(part 1 of 2)
# Autodesk Inventor assembly: 110033226_iam_04_大橋塔樓
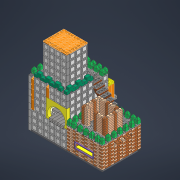
[picture p0: Inventor's stored thumbnail of the model, 180x180]
Saved by Autodesk Inventor 2022 (Build 260153000, 153)
## iProperties
Created: 2022-06-23
Part Number: 110033226_iam_04_大橋塔樓
Document SubType Name: Assembly
Designer: User
Author: User
## Documents named in this file (16)
- D:\D-disk\pomelo\大一\下學期\機械設計製圖\1100332260_LEGOproj_沒有公主城堡\110033226_iam_04_大橋塔樓.iam
- D:\D-disk\pomelo\大一\下學期\機械設計製圖\1100332260_LEGOproj_沒有公主城堡\110033226_ipt_07_磚塊樺木(2x1).ipt
- D:\D-disk\pomelo\大一\下學期\機械設計製圖\1100332260_LEGOproj_沒有公主城堡\110033226_ipt_05_房子底座.ipt
- D:\D-disk\pomelo\大一\下學期\機械設計製圖\1100332260_LEGOproj_沒有公主城堡\110033226_ipt_06_磚塊樺木(1x1).ipt
- D:\D-disk\pomelo\大一\下學期\機械設計製圖\1100332260_LEGOproj_沒有公主城堡\110033226_ipt_16_圍牆.ipt
- D:\D-disk\pomelo\大一\下學期\機械設計製圖\1100332260_LEGOproj_沒有公主城堡\110033226_ipt_08_平滑面(3x1).ipt
- D:\D-disk\pomelo\大一\下學期\機械設計製圖\1100332260_LEGOproj_沒有公主城堡\110033226_ipt_20_塔樓窗戶.ipt
- D:\D-disk\pomelo\大一\下學期\機械設計製圖\1100332260_LEGOproj_沒有公主城堡\110033226_ipt_21_柵欄.ipt
- D:\D-disk\pomelo\大一\下學期\機械設計製圖\1100332260_LEGOproj_沒有公主城堡\110033226_ipt_11_樓梯支架.ipt
- D:\D-disk\pomelo\大一\下學期\機械設計製圖\1100332260_LEGOproj_沒有公主城堡\110033226_ipt_22_塔樓牆壁.ipt
- D:\D-disk\pomelo\大一\下學期\機械設計製圖\1100332260_LEGOproj_沒有公主城堡\110033226_ipt_23_塔樓門口.ipt
- D:\D-disk\pomelo\大一\下學期\機械設計製圖\1100332260_LEGOproj_沒有公主城堡\110033226_ipt_10_木板條.ipt
- D:\D-disk\pomelo\大一\下學期\機械設計製圖\1100332260_LEGOproj_沒有公主城堡\110033226_ipt_24_直條(3x1).ipt
- D:\D-disk\pomelo\大一\下學期\機械設計製圖\1100332260_LEGOproj_沒有公主城堡\110033226_ipt_25_塔樓大窗戶.ipt
- D:\D-disk\pomelo\大一\下學期\機械設計製圖\1100332260_LEGOproj_沒有公主城堡\110033226_ipt_12_平滑面(2x1).ipt
- D:\D-disk\pomelo\大一\下學期\機械設計製圖\1100332260_LEGOproj_沒有公主城堡\110033226_ipt_18_大橋圍牆.ipt
## Components (1135 placed, 15 different names)
1. 110033226_ipt_05_房子底座:1 — 貼合:1, 貼合:2, 貼合:3, 貼合:4, 貼合:5, 貼合:13, 貼合:14, 貼合:15, 貼合:16, 貼合:17, 貼合:96, 貼合:97
2. 110033226_ipt_07_磚塊樺木(2x1):1 — 貼合:28, 貼合:29, 貼合:30, 貼合:148
3. 110033226_ipt_20_塔樓窗戶:1 — 貼合:37, 貼合:38, 貼合:39, 貼合:40
4. 110033226_ipt_20_塔樓窗戶:2 — 貼合:41, 貼合:42, 貼合:43
5. 110033226_ipt_08_平滑面(3x1):58 — 貼合:69, 貼合:70, 貼合:71, 貼合:193, 貼合:194, 貼合:195, 貼合:202, 貼合:204
6. 110033226_ipt_08_平滑面(3x1):59 — 貼合:72, 貼合:73, 貼合:74
7. 110033226_ipt_08_平滑面(3x1):60 — 貼合:75, 貼合:82, 貼合:83
8. 110033226_ipt_08_平滑面(3x1):61 — 貼合:76, 貼合:84, 貼合:85
9. 110033226_ipt_08_平滑面(3x1):62 — 貼合:78, 貼合:86, 貼合:87
10. 110033226_ipt_08_平滑面(3x1):63 — 貼合:80, 貼合:94, 貼合:95
11. 110033226_ipt_08_平滑面(3x1):64 — 貼合:77, 貼合:88, 貼合:89
12. 110033226_ipt_08_平滑面(3x1):65 — 貼合:79, 貼合:90, 貼合:91
13. 110033226_ipt_08_平滑面(3x1):66 — 貼合:81, 貼合:92, 貼合:93
14. 110033226_ipt_05_房子底座:2 — 貼合:96, 貼合:97, 貼合:98, 貼合:99, 貼合:100, 貼合:101, 對稱:1, 貼合:102, 貼合:103, 貼合:137, 貼合:138, 貼合:139, 貼合:143, 貼合:144, 貼合:145, 貼合:146, 貼合:147, 貼合:170
15. 110033226_ipt_23_塔樓門口:1 — 貼合:104, 貼合:105, 貼合:106, 貼合:179, 貼合:180, 貼合:181, 貼合:182, 貼合:183
16. 110033226_ipt_10_木板條:1 — 貼合:134, 貼合:135, 貼合:136
17. 110033226_ipt_10_木板條:33 — 貼合:128, 貼合:129, 貼合:130
18. 110033226_ipt_10_木板條:34 — 貼合:113, 貼合:114, 貼合:115, 貼合:116, 貼合:117, 貼合:118
19. 110033226_ipt_10_木板條:35 — 貼合:140, 貼合:141, 貼合:142
20. 110033226_ipt_10_木板條:36 — 貼合:131, 貼合:132, 貼合:133
21. 110033226_ipt_10_木板條:42 — 貼合:119, 貼合:120, 貼合:121
22. 110033226_ipt_24_直條(3x1):8 — 貼合:182, 貼合:183
23. 110033226_ipt_25_塔樓大窗戶:1 — 貼合:196, 貼合:197, 貼合:198
24. 110033226_ipt_16_圍牆:1 — 貼合:25, 貼合:26, 貼合:27
25. 110033226_ipt_16_圍牆:2
26. 110033226_ipt_21_柵欄:1 — 貼合:44, 貼合:45, 貼合:46, 貼合:48
27. 110033226_ipt_21_柵欄:4
28. 110033226_ipt_21_柵欄:5
29. 110033226_ipt_21_柵欄:6
30. 110033226_ipt_21_柵欄:7
31. 110033226_ipt_21_柵欄:8
32. 110033226_ipt_21_柵欄:9
33. 110033226_ipt_21_柵欄:14
34. 110033226_ipt_21_柵欄:15
35. 110033226_ipt_21_柵欄:16
36. 110033226_ipt_21_柵欄:17
37. 110033226_ipt_21_柵欄:18
38. 110033226_ipt_21_柵欄:19
39. 110033226_ipt_21_柵欄:20
40. 110033226_ipt_21_柵欄:2 — 貼合:47, 貼合:48, 貼合:49
41. 110033226_ipt_21_柵欄:10
42. 110033226_ipt_21_柵欄:11
43. 110033226_ipt_21_柵欄:12
44. 110033226_ipt_21_柵欄:13
45. 110033226_ipt_21_柵欄:21
46. 110033226_ipt_21_柵欄:22
47. 110033226_ipt_21_柵欄:23
48. 110033226_ipt_21_柵欄:24
49. 110033226_ipt_21_柵欄:25
50. 110033226_ipt_22_塔樓牆壁:2 — 對稱:1, 貼合:102, 貼合:103
51. 110033226_ipt_22_塔樓牆壁:22
52. 110033226_ipt_22_塔樓牆壁:23
53. 110033226_ipt_22_塔樓牆壁:24
54. 110033226_ipt_22_塔樓牆壁:25
55. 110033226_ipt_22_塔樓牆壁:26
56. 110033226_ipt_22_塔樓牆壁:27
57. 110033226_ipt_22_塔樓牆壁:28
58. 110033226_ipt_22_塔樓牆壁:29
59. 110033226_ipt_22_塔樓牆壁:30
60. 110033226_ipt_22_塔樓牆壁:31
61. 110033226_ipt_22_塔樓牆壁:32
62. 110033226_ipt_22_塔樓牆壁:33
63. 110033226_ipt_22_塔樓牆壁:34
64. 110033226_ipt_22_塔樓牆壁:35
65. 110033226_ipt_22_塔樓牆壁:36
66. 110033226_ipt_22_塔樓牆壁:37
67. 110033226_ipt_22_塔樓牆壁:38
68. 110033226_ipt_22_塔樓牆壁:39
69. 110033226_ipt_22_塔樓牆壁:40
70. 110033226_ipt_22_塔樓牆壁:41 — 貼合:171, 貼合:172
71. 110033226_ipt_22_塔樓牆壁:42
72. 110033226_ipt_22_塔樓牆壁:43
73. 110033226_ipt_22_塔樓牆壁:44
74. 110033226_ipt_22_塔樓牆壁:45 — 貼合:173, 貼合:174, 貼合:175
75. 110033226_ipt_22_塔樓牆壁:46 — 貼合:107, 貼合:108, 貼合:109
76. 110033226_ipt_22_塔樓牆壁:48
77. 110033226_ipt_22_塔樓牆壁:49
78. 110033226_ipt_22_塔樓牆壁:50
79. 110033226_ipt_22_塔樓牆壁:51 — 貼合:215
80. 110033226_ipt_22_塔樓牆壁:52
81. 110033226_ipt_22_塔樓牆壁:53
82. 110033226_ipt_22_塔樓牆壁:54
83. 110033226_ipt_22_塔樓牆壁:215
84. 110033226_ipt_22_塔樓牆壁:216 — 貼合:213, 貼合:214
85. 110033226_ipt_11_樓梯支架:41 — 貼合:113, 貼合:114, 貼合:118, 貼合:119, 貼合:121
86. 110033226_ipt_11_樓梯支架:42 — 貼合:120
87. 110033226_ipt_11_樓梯支架:43 — 貼合:134
88. 110033226_ipt_11_樓梯支架:44 — 貼合:135, 貼合:136
89. 110033226_ipt_11_樓梯支架:45 — 貼合:123
90. 110033226_ipt_11_樓梯支架:46 — 貼合:122, 貼合:124
91. 110033226_ipt_10_木板條:3 — 貼合:122, 貼合:123, 貼合:124
92. 110033226_ipt_10_木板條:43
93. 110033226_ipt_10_木板條:44 — 貼合:125, 貼合:126, 貼合:127
94. 110033226_ipt_11_樓梯支架:40 — 貼合:125, 貼合:126, 貼合:127, 貼合:142
95. 110033226_ipt_11_樓梯支架:47 — 貼合:140, 貼合:141
96. 110033226_ipt_11_樓梯支架:48 — 貼合:131, 貼合:133
97. 110033226_ipt_11_樓梯支架:49 — 貼合:132
98. 110033226_ipt_11_樓梯支架:50 — 貼合:129
99. 110033226_ipt_11_樓梯支架:51 — 貼合:128, 貼合:130
100. 110033226_ipt_10_木板條:39 — 貼合:137, 貼合:138, 貼合:139
101. 110033226_ipt_10_木板條:45
102. 110033226_ipt_22_塔樓牆壁:55 — 貼合:143, 貼合:144, 貼合:145, 對稱:2, 貼合:152, 貼合:153
103. 110033226_ipt_22_塔樓牆壁:140
104. 110033226_ipt_22_塔樓牆壁:141
105. 110033226_ipt_22_塔樓牆壁:142 — 貼合:196
106. 110033226_ipt_22_塔樓牆壁:143
107. 110033226_ipt_22_塔樓牆壁:144
108. 110033226_ipt_22_塔樓牆壁:145 — 貼合:149, 貼合:150, 貼合:151
109. 110033226_ipt_22_塔樓牆壁:147 — 貼合:149, 貼合:150, 貼合:151, 貼合:198
110. 110033226_ipt_22_塔樓牆壁:149
111. 110033226_ipt_22_塔樓牆壁:148 — 對稱:2, 貼合:152, 貼合:153
112. 110033226_ipt_22_塔樓牆壁:150
113. 110033226_ipt_22_塔樓牆壁:151 — 貼合:178
114. 110033226_ipt_22_塔樓牆壁:152
115. 110033226_ipt_22_塔樓牆壁:153
116. 110033226_ipt_22_塔樓牆壁:154
117. 110033226_ipt_22_塔樓牆壁:155
118. 110033226_ipt_22_塔樓牆壁:156
119. 110033226_ipt_22_塔樓牆壁:157
120. 110033226_ipt_22_塔樓牆壁:158 — 貼合:197
121. 110033226_ipt_22_塔樓牆壁:159
122. 110033226_ipt_22_塔樓牆壁:160
123. 110033226_ipt_22_塔樓牆壁:161 — 貼合:199, 貼合:200, 貼合:201
124. 110033226_ipt_22_塔樓牆壁:162 — 貼合:205
125. 110033226_ipt_07_磚塊樺木(2x1):234 — 對稱:3, 貼合:163, 貼合:164, 貼合:165, 貼合:166, 貼合:167
126. 110033226_ipt_06_磚塊樺木(1x1):234 — 貼合:165, 貼合:166, 貼合:167
127. 110033226_ipt_07_磚塊樺木(2x1):235
128. 110033226_ipt_06_磚塊樺木(1x1):235
129. 110033226_ipt_07_磚塊樺木(2x1):236
130. 110033226_ipt_06_磚塊樺木(1x1):236
131. 110033226_ipt_07_磚塊樺木(2x1):237
132. 110033226_ipt_06_磚塊樺木(1x1):237
133. 110033226_ipt_07_磚塊樺木(2x1):238
134. 110033226_ipt_06_磚塊樺木(1x1):238
135. 110033226_ipt_07_磚塊樺木(2x1):239
136. 110033226_ipt_06_磚塊樺木(1x1):239
137. 110033226_ipt_07_磚塊樺木(2x1):240
138. 110033226_ipt_06_磚塊樺木(1x1):240
139. 110033226_ipt_07_磚塊樺木(2x1):241
140. 110033226_ipt_06_磚塊樺木(1x1):241
141. 110033226_ipt_07_磚塊樺木(2x1):242
142. 110033226_ipt_06_磚塊樺木(1x1):242
143. 110033226_ipt_07_磚塊樺木(2x1):243
144. 110033226_ipt_06_磚塊樺木(1x1):243
145. 110033226_ipt_07_磚塊樺木(2x1):244
146. 110033226_ipt_06_磚塊樺木(1x1):244
147. 110033226_ipt_07_磚塊樺木(2x1):245
148. 110033226_ipt_06_磚塊樺木(1x1):245
149. 110033226_ipt_07_磚塊樺木(2x1):246
150. 110033226_ipt_06_磚塊樺木(1x1):246
151. 110033226_ipt_07_磚塊樺木(2x1):247
152. 110033226_ipt_06_磚塊樺木(1x1):247
153. 110033226_ipt_07_磚塊樺木(2x1):248
154. 110033226_ipt_06_磚塊樺木(1x1):248
155. 110033226_ipt_07_磚塊樺木(2x1):249
156. 110033226_ipt_06_磚塊樺木(1x1):249
157. 110033226_ipt_07_磚塊樺木(2x1):250
158. 110033226_ipt_06_磚塊樺木(1x1):250
159. 110033226_ipt_07_磚塊樺木(2x1):251
160. 110033226_ipt_06_磚塊樺木(1x1):251
161. 110033226_ipt_07_磚塊樺木(2x1):252
162. 110033226_ipt_06_磚塊樺木(1x1):252
163. 110033226_ipt_07_磚塊樺木(2x1):253
164. 110033226_ipt_06_磚塊樺木(1x1):253
165. 110033226_ipt_07_磚塊樺木(2x1):228 — 貼合:57, 貼合:58, 貼合:59, 貼合:61, 貼合:62
166. 110033226_ipt_06_磚塊樺木(1x1):229 — 貼合:60, 貼合:61, 貼合:62
167. 110033226_ipt_07_磚塊樺木(2x1):254
168. 110033226_ipt_06_磚塊樺木(1x1):254
169. 110033226_ipt_07_磚塊樺木(2x1):259
170. 110033226_ipt_06_磚塊樺木(1x1):259
171. 110033226_ipt_07_磚塊樺木(2x1):264
172. 110033226_ipt_06_磚塊樺木(1x1):264
173. 110033226_ipt_07_磚塊樺木(2x1):269
174. 110033226_ipt_06_磚塊樺木(1x1):269
175. 110033226_ipt_07_磚塊樺木(2x1):274
176. 110033226_ipt_06_磚塊樺木(1x1):274
177. 110033226_ipt_07_磚塊樺木(2x1):279
178. 110033226_ipt_06_磚塊樺木(1x1):279
179. 110033226_ipt_07_磚塊樺木(2x1):284
180. 110033226_ipt_06_磚塊樺木(1x1):284
181. 110033226_ipt_07_磚塊樺木(2x1):289
182. 110033226_ipt_06_磚塊樺木(1x1):289
183. 110033226_ipt_07_磚塊樺木(2x1):294
184. 110033226_ipt_06_磚塊樺木(1x1):294
185. 110033226_ipt_06_磚塊樺木(1x1):299 — 對稱:4, 貼合:168, 貼合:169
186. 110033226_ipt_06_磚塊樺木(1x1):300
187. 110033226_ipt_06_磚塊樺木(1x1):301
188. 110033226_ipt_06_磚塊樺木(1x1):302
189. 110033226_ipt_06_磚塊樺木(1x1):303
190. 110033226_ipt_06_磚塊樺木(1x1):304
191. 110033226_ipt_06_磚塊樺木(1x1):305
192. 110033226_ipt_06_磚塊樺木(1x1):306
193. 110033226_ipt_06_磚塊樺木(1x1):307
194. 110033226_ipt_06_磚塊樺木(1x1):308
195. 110033226_ipt_24_直條(3x1):1 — 貼合:170, 貼合:171, 貼合:172
196. 110033226_ipt_24_直條(3x1):2
197. 110033226_ipt_24_直條(3x1):3
198. 110033226_ipt_24_直條(3x1):4
199. 110033226_ipt_22_塔樓牆壁:194 — 貼合:173, 貼合:174, 貼合:175
200. 110033226_ipt_22_塔樓牆壁:206
201. 110033226_ipt_22_塔樓牆壁:207
202. 110033226_ipt_22_塔樓牆壁:208 — 貼合:184
203. 110033226_ipt_22_塔樓牆壁:209 — 貼合:185, 貼合:186
204. 110033226_ipt_24_直條(3x1):5 — 貼合:176, 貼合:177, 貼合:178
205. 110033226_ipt_24_直條(3x1):6
206. 110033226_ipt_24_直條(3x1):7
207. 110033226_ipt_22_塔樓牆壁:193 — 貼合:179, 貼合:180, 貼合:181
208. 110033226_ipt_22_塔樓牆壁:210
209. 110033226_ipt_22_塔樓牆壁:211
210. 110033226_ipt_22_塔樓牆壁:212
211. 110033226_ipt_22_塔樓牆壁:213
212. 110033226_ipt_22_塔樓牆壁:214
213. 110033226_ipt_22_塔樓牆壁:217 — 貼合:184, 貼合:185, 貼合:186
214. 110033226_ipt_22_塔樓牆壁:218
215. 110033226_ipt_22_塔樓牆壁:219
216. 110033226_ipt_22_塔樓牆壁:220
217. 110033226_ipt_22_塔樓牆壁:221
218. 110033226_ipt_22_塔樓牆壁:222 — 貼合:218
219. 110033226_ipt_22_塔樓牆壁:223
220. 110033226_ipt_22_塔樓牆壁:224 — 貼合:216, 貼合:217
221. 110033226_ipt_22_塔樓牆壁:225 — 貼合:187, 貼合:188, 貼合:189
222. 110033226_ipt_22_塔樓牆壁:226 — 貼合:190, 貼合:191, 貼合:192
223. 110033226_ipt_21_柵欄:26 — 貼合:190, 貼合:191, 貼合:192
224. 110033226_ipt_21_柵欄:27
225. 110033226_ipt_21_柵欄:28
226. 110033226_ipt_21_柵欄:29
227. 110033226_ipt_21_柵欄:30
228. 110033226_ipt_21_柵欄:31
229. 110033226_ipt_21_柵欄:32
230. 110033226_ipt_21_柵欄:33
231. 110033226_ipt_21_柵欄:34
232. 110033226_ipt_21_柵欄:35
233. 110033226_ipt_21_柵欄:36
234. 110033226_ipt_21_柵欄:37
235. 110033226_ipt_08_平滑面(3x1):67 — 貼合:193, 貼合:194, 貼合:195
236. 110033226_ipt_08_平滑面(3x1):70 — 貼合:203
237. 110033226_ipt_08_平滑面(3x1):71 — 貼合:208, 貼合:222, 貼合:223, 貼合:224
238. 110033226_ipt_08_平滑面(3x1):72
239. 110033226_ipt_08_平滑面(3x1):73 — 貼合:225, 貼合:226
240. 110033226_ipt_08_平滑面(3x1):74
241. 110033226_ipt_08_平滑面(3x1):75
242. 110033226_ipt_08_平滑面(3x1):76 — 貼合:227
243. 110033226_ipt_08_平滑面(3x1):77
244. 110033226_ipt_08_平滑面(3x1):78
245. 110033226_ipt_08_平滑面(3x1):79
246. 110033226_ipt_08_平滑面(3x1):80
247. 110033226_ipt_08_平滑面(3x1):81
248. 110033226_ipt_08_平滑面(3x1):82
249. 110033226_ipt_08_平滑面(3x1):83
250. 110033226_ipt_08_平滑面(3x1):84
251. 110033226_ipt_08_平滑面(3x1):85
252. 110033226_ipt_08_平滑面(3x1):86
253. 110033226_ipt_08_平滑面(3x1):87
254. 110033226_ipt_08_平滑面(3x1):88
255. 110033226_ipt_08_平滑面(3x1):89
256. 110033226_ipt_08_平滑面(3x1):90
257. 110033226_ipt_08_平滑面(3x1):91 — 貼合:228, 貼合:229, 貼合:230
258. 110033226_ipt_08_平滑面(3x1):92
259. 110033226_ipt_08_平滑面(3x1):93
260. 110033226_ipt_08_平滑面(3x1):94
261. 110033226_ipt_08_平滑面(3x1):95 — 貼合:206
262. 110033226_ipt_08_平滑面(3x1):96
263. 110033226_ipt_08_平滑面(3x1):97
264. 110033226_ipt_08_平滑面(3x1):98 — 貼合:207
265. 110033226_ipt_22_塔樓牆壁:227 — 貼合:199, 貼合:200, 貼合:201
266. 110033226_ipt_22_塔樓牆壁:229
267. 110033226_ipt_22_塔樓牆壁:230
268. 110033226_ipt_22_塔樓牆壁:231
269. 110033226_ipt_22_塔樓牆壁:232
270. 110033226_ipt_22_塔樓牆壁:233
271. 110033226_ipt_22_塔樓牆壁:234
272. 110033226_ipt_22_塔樓牆壁:235 — 貼合:211, 貼合:212
273. 110033226_ipt_08_平滑面(3x1):100 — 貼合:202, 貼合:203, 貼合:204
274. 110033226_ipt_08_平滑面(3x1):102 — 貼合:210
275. 110033226_ipt_08_平滑面(3x1):101 — 貼合:205, 貼合:206, 貼合:207
276. 110033226_ipt_08_平滑面(3x1):103
277. 110033226_ipt_08_平滑面(3x1):104 — 貼合:209, 貼合:220
278. 110033226_ipt_08_平滑面(3x1):105
279. 110033226_ipt_08_平滑面(3x1):106
280. 110033226_ipt_08_平滑面(3x1):107
281. 110033226_ipt_12_平滑面(2x1):1 — 貼合:208, 貼合:209, 貼合:210, 貼合:219, 貼合:221
282. 110033226_ipt_12_平滑面(2x1):3
283. 110033226_ipt_21_柵欄:42 — 貼合:211, 貼合:212
284. 110033226_ipt_21_柵欄:43
285. 110033226_ipt_21_柵欄:44
286. 110033226_ipt_21_柵欄:45
287. 110033226_ipt_21_柵欄:46
288. 110033226_ipt_21_柵欄:47
289. 110033226_ipt_21_柵欄:48
290. 110033226_ipt_21_柵欄:49
291. 110033226_ipt_21_柵欄:50
292. 110033226_ipt_21_柵欄:51
293. 110033226_ipt_21_柵欄:52
294. 110033226_ipt_21_柵欄:53
295. 110033226_ipt_18_大橋圍牆:2 — 貼合:213, 貼合:214, 貼合:215
296. 110033226_ipt_18_大橋圍牆:3
297. 110033226_ipt_18_大橋圍牆:4
298. 110033226_ipt_18_大橋圍牆:1 — 貼合:216, 貼合:217, 貼合:218
299. 110033226_ipt_18_大橋圍牆:5
300. 110033226_ipt_18_大橋圍牆:6
301. 110033226_ipt_12_平滑面(2x1):4 — 貼合:234, 貼合:235, 貼合:236
302. 110033226_ipt_12_平滑面(2x1):8
303. 110033226_ipt_12_平滑面(2x1):9
304. 110033226_ipt_12_平滑面(2x1):10
305. 110033226_ipt_12_平滑面(2x1):11
306. 110033226_ipt_12_平滑面(2x1):12
307. 110033226_ipt_12_平滑面(2x1):13
308. 110033226_ipt_12_平滑面(2x1):14
309. 110033226_ipt_12_平滑面(2x1):15
310. 110033226_ipt_12_平滑面(2x1):16
311. 110033226_ipt_12_平滑面(2x1):17
312. 110033226_ipt_12_平滑面(2x1):18
313. 110033226_ipt_12_平滑面(2x1):19
314. 110033226_ipt_12_平滑面(2x1):20
315. 110033226_ipt_12_平滑面(2x1):21
316. 110033226_ipt_12_平滑面(2x1):22
317. 110033226_ipt_12_平滑面(2x1):23
318. 110033226_ipt_12_平滑面(2x1):24
319. 110033226_ipt_12_平滑面(2x1):25
320. 110033226_ipt_12_平滑面(2x1):26
321. 110033226_ipt_12_平滑面(2x1):27
322. 110033226_ipt_12_平滑面(2x1):28
323. 110033226_ipt_12_平滑面(2x1):29
324. 110033226_ipt_12_平滑面(2x1):30
325. 110033226_ipt_12_平滑面(2x1):31
326. 110033226_ipt_12_平滑面(2x1):32
327. 110033226_ipt_12_平滑面(2x1):33
328. 110033226_ipt_12_平滑面(2x1):34
329. 110033226_ipt_22_塔樓牆壁:298 — 貼合:237, 貼合:238, 貼合:239
330. 110033226_ipt_22_塔樓牆壁:299
331. 110033226_ipt_22_塔樓牆壁:300
332. 110033226_ipt_12_平滑面(2x1):35
333. 110033226_ipt_12_平滑面(2x1):36
334. 110033226_ipt_12_平滑面(2x1):37
335. 110033226_ipt_12_平滑面(2x1):38
336. 110033226_ipt_12_平滑面(2x1):39
337. 110033226_ipt_12_平滑面(2x1):40
338. 110033226_ipt_12_平滑面(2x1):41
339. 110033226_ipt_12_平滑面(2x1):42
340. 110033226_ipt_12_平滑面(2x1):43
341. 110033226_ipt_12_平滑面(2x1):44
342. 110033226_ipt_12_平滑面(2x1):45
343. 110033226_ipt_12_平滑面(2x1):46
344. 110033226_ipt_12_平滑面(2x1):47
345. 110033226_ipt_12_平滑面(2x1):48
346. 110033226_ipt_06_磚塊樺木(1x1):2 — 貼合:22, 貼合:23, 貼合:24
347. 110033226_ipt_07_磚塊樺木(2x1):2 — 貼合:19, 貼合:20, 貼合:21, 貼合:23
348. 110033226_ipt_06_磚塊樺木(1x1):1 — 貼合:16, 貼合:17, 貼合:18, 貼合:19, 貼合:21
349. 110033226_ipt_07_磚塊樺木(2x1):5 — 貼合:13, 貼合:14, 貼合:15, 貼合:18, 貼合:20, 貼合:22, 貼合:24
350. 110033226_ipt_06_磚塊樺木(1x1):60
351. 110033226_ipt_07_磚塊樺木(2x1):61
352. 110033226_ipt_06_磚塊樺木(1x1):61
353. 110033226_ipt_07_磚塊樺木(2x1):62
354. 110033226_ipt_06_磚塊樺木(1x1):62
355. 110033226_ipt_07_磚塊樺木(2x1):63
356. 110033226_ipt_06_磚塊樺木(1x1):63
357. 110033226_ipt_07_磚塊樺木(2x1):64
358. 110033226_ipt_06_磚塊樺木(1x1):64
359. 110033226_ipt_07_磚塊樺木(2x1):65
360. 110033226_ipt_06_磚塊樺木(1x1):65
361. 110033226_ipt_07_磚塊樺木(2x1):66
362. 110033226_ipt_06_磚塊樺木(1x1):66
363. 110033226_ipt_07_磚塊樺木(2x1):67
364. 110033226_ipt_06_磚塊樺木(1x1):67
365. 110033226_ipt_07_磚塊樺木(2x1):68
366. 110033226_ipt_06_磚塊樺木(1x1):68
367. 110033226_ipt_07_磚塊樺木(2x1):69
368. 110033226_ipt_06_磚塊樺木(1x1):69
369. 110033226_ipt_07_磚塊樺木(2x1):70
370. 110033226_ipt_06_磚塊樺木(1x1):70
371. 110033226_ipt_07_磚塊樺木(2x1):71
372. 110033226_ipt_06_磚塊樺木(1x1):71
373. 110033226_ipt_07_磚塊樺木(2x1):72
374. 110033226_ipt_06_磚塊樺木(1x1):72
375. 110033226_ipt_07_磚塊樺木(2x1):73
376. 110033226_ipt_06_磚塊樺木(1x1):73
377. 110033226_ipt_07_磚塊樺木(2x1):74
378. 110033226_ipt_06_磚塊樺木(1x1):74
379. 110033226_ipt_07_磚塊樺木(2x1):75
380. 110033226_ipt_06_磚塊樺木(1x1):75
381. 110033226_ipt_07_磚塊樺木(2x1):76
382. 110033226_ipt_06_磚塊樺木(1x1):76
383. 110033226_ipt_07_磚塊樺木(2x1):77
384. 110033226_ipt_06_磚塊樺木(1x1):77
385. 110033226_ipt_07_磚塊樺木(2x1):78
386. 110033226_ipt_06_磚塊樺木(1x1):78
387. 110033226_ipt_07_磚塊樺木(2x1):79
388. 110033226_ipt_06_磚塊樺木(1x1):79
389. 110033226_ipt_07_磚塊樺木(2x1):80
390. 110033226_ipt_06_磚塊樺木(1x1):80
391. 110033226_ipt_07_磚塊樺木(2x1):81
392. 110033226_ipt_06_磚塊樺木(1x1):81
393. 110033226_ipt_07_磚塊樺木(2x1):82
394. 110033226_ipt_06_磚塊樺木(1x1):82
395. 110033226_ipt_07_磚塊樺木(2x1):83
396. 110033226_ipt_06_磚塊樺木(1x1):83
397. 110033226_ipt_07_磚塊樺木(2x1):84
398. 110033226_ipt_06_磚塊樺木(1x1):84
399. 110033226_ipt_07_磚塊樺木(2x1):85
400. 110033226_ipt_06_磚塊樺木(1x1):85
401. 110033226_ipt_07_磚塊樺木(2x1):86
402. 110033226_ipt_06_磚塊樺木(1x1):86
403. 110033226_ipt_07_磚塊樺木(2x1):87
404. 110033226_ipt_06_磚塊樺木(1x1):87
405. 110033226_ipt_07_磚塊樺木(2x1):88
406. 110033226_ipt_06_磚塊樺木(1x1):88
407. 110033226_ipt_07_磚塊樺木(2x1):89
408. 110033226_ipt_06_磚塊樺木(1x1):89
409. 110033226_ipt_07_磚塊樺木(2x1):90
410. 110033226_ipt_06_磚塊樺木(1x1):90
411. 110033226_ipt_07_磚塊樺木(2x1):91
412. 110033226_ipt_06_磚塊樺木(1x1):91
413. 110033226_ipt_07_磚塊樺木(2x1):92
414. 110033226_ipt_06_磚塊樺木(1x1):92
415. 110033226_ipt_07_磚塊樺木(2x1):93
416. 110033226_ipt_06_磚塊樺木(1x1):93
417. 110033226_ipt_07_磚塊樺木(2x1):94
418. 110033226_ipt_06_磚塊樺木(1x1):94
419. 110033226_ipt_07_磚塊樺木(2x1):95
420. 110033226_ipt_06_磚塊樺木(1x1):95
421. 110033226_ipt_07_磚塊樺木(2x1):96
422. 110033226_ipt_06_磚塊樺木(1x1):96
423. 110033226_ipt_07_磚塊樺木(2x1):97
424. 110033226_ipt_06_磚塊樺木(1x1):97
425. 110033226_ipt_07_磚塊樺木(2x1):98
426. 110033226_ipt_06_磚塊樺木(1x1):98
427. 110033226_ipt_07_磚塊樺木(2x1):99
428. 110033226_ipt_06_磚塊樺木(1x1):99
429. 110033226_ipt_07_磚塊樺木(2x1):100
430. 110033226_ipt_06_磚塊樺木(1x1):104
431. 110033226_ipt_07_磚塊樺木(2x1):105
432. 110033226_ipt_06_磚塊樺木(1x1):105
433. 110033226_ipt_07_磚塊樺木(2x1):106
434. 110033226_ipt_06_磚塊樺木(1x1):106
435. 110033226_ipt_07_磚塊樺木(2x1):107
436. 110033226_ipt_06_磚塊樺木(1x1):107
437. 110033226_ipt_07_磚塊樺木(2x1):108
438. 110033226_ipt_06_磚塊樺木(1x1):108
439. 110033226_ipt_07_磚塊樺木(2x1):109
440. 110033226_ipt_06_磚塊樺木(1x1):109
441. 110033226_ipt_07_磚塊樺木(2x1):110
442. 110033226_ipt_06_磚塊樺木(1x1):110
443. 110033226_ipt_07_磚塊樺木(2x1):111
444. 110033226_ipt_06_磚塊樺木(1x1):111
445. 110033226_ipt_07_磚塊樺木(2x1):112
446. 110033226_ipt_06_磚塊樺木(1x1):112
447. 110033226_ipt_07_磚塊樺木(2x1):113
448. 110033226_ipt_06_磚塊樺木(1x1):113
449. 110033226_ipt_07_磚塊樺木(2x1):114
450. 110033226_ipt_06_磚塊樺木(1x1):114
451. 110033226_ipt_07_磚塊樺木(2x1):115
452. 110033226_ipt_06_磚塊樺木(1x1):115
453. 110033226_ipt_07_磚塊樺木(2x1):116
454. 110033226_ipt_06_磚塊樺木(1x1):116
455. 110033226_ipt_07_磚塊樺木(2x1):117
456. 110033226_ipt_06_磚塊樺木(1x1):117 — 貼合:98
457. 110033226_ipt_07_磚塊樺木(2x1):118
458. 110033226_ipt_06_磚塊樺木(1x1):118
459. 110033226_ipt_07_磚塊樺木(2x1):119
460. 110033226_ipt_06_磚塊樺木(1x1):119
461. 110033226_ipt_07_磚塊樺木(2x1):120
462. 110033226_ipt_06_磚塊樺木(1x1):120
463. 110033226_ipt_07_磚塊樺木(2x1):121
464. 110033226_ipt_06_磚塊樺木(1x1):121
465. 110033226_ipt_07_磚塊樺木(2x1):122
466. 110033226_ipt_06_磚塊樺木(1x1):122
467. 110033226_ipt_07_磚塊樺木(2x1):123
468. 110033226_ipt_06_磚塊樺木(1x1):123
469. 110033226_ipt_07_磚塊樺木(2x1):124
470. 110033226_ipt_06_磚塊樺木(1x1):124
471. 110033226_ipt_07_磚塊樺木(2x1):125
472. 110033226_ipt_06_磚塊樺木(1x1):125
473. 110033226_ipt_07_磚塊樺木(2x1):126
474. 110033226_ipt_06_磚塊樺木(1x1):126
475. 110033226_ipt_07_磚塊樺木(2x1):127
476. 110033226_ipt_06_磚塊樺木(1x1):127
477. 110033226_ipt_07_磚塊樺木(2x1):128
478. 110033226_ipt_06_磚塊樺木(1x1):128
479. 110033226_ipt_07_磚塊樺木(2x1):129
480. 110033226_ipt_06_磚塊樺木(1x1):129
481. 110033226_ipt_07_磚塊樺木(2x1):130
482. 110033226_ipt_06_磚塊樺木(1x1):130
483. 110033226_ipt_07_磚塊樺木(2x1):131
484. 110033226_ipt_06_磚塊樺木(1x1):131
485. 110033226_ipt_07_磚塊樺木(2x1):132
486. 110033226_ipt_06_磚塊樺木(1x1):132
487. 110033226_ipt_07_磚塊樺木(2x1):133
488. 110033226_ipt_06_磚塊樺木(1x1):133
489. 110033226_ipt_07_磚塊樺木(2x1):134
490. 110033226_ipt_06_磚塊樺木(1x1):134
491. 110033226_ipt_07_磚塊樺木(2x1):135
492. 110033226_ipt_06_磚塊樺木(1x1):135
493. 110033226_ipt_07_磚塊樺木(2x1):136
494. 110033226_ipt_06_磚塊樺木(1x1):136
495. 110033226_ipt_07_磚塊樺木(2x1):137
496. 110033226_ipt_06_磚塊樺木(1x1):137
497. 110033226_ipt_07_磚塊樺木(2x1):138
498. 110033226_ipt_06_磚塊樺木(1x1):138
499. 110033226_ipt_07_磚塊樺木(2x1):139
500. 110033226_ipt_06_磚塊樺木(1x1):139
501. 110033226_ipt_07_磚塊樺木(2x1):140
502. 110033226_ipt_06_磚塊樺木(1x1):140
503. 110033226_ipt_07_磚塊樺木(2x1):141
504. 110033226_ipt_06_磚塊樺木(1x1):141
505. 110033226_ipt_07_磚塊樺木(2x1):142
506. 110033226_ipt_06_磚塊樺木(1x1):142
507. 110033226_ipt_07_磚塊樺木(2x1):143
508. 110033226_ipt_06_磚塊樺木(1x1):143
509. 110033226_ipt_07_磚塊樺木(2x1):144
510. 110033226_ipt_06_磚塊樺木(1x1):144
511. 110033226_ipt_07_磚塊樺木(2x1):145
512. 110033226_ipt_06_磚塊樺木(1x1):145
513. 110033226_ipt_07_磚塊樺木(2x1):146
514. 110033226_ipt_06_磚塊樺木(1x1):146
515. 110033226_ipt_07_磚塊樺木(2x1):147
516. 110033226_ipt_06_磚塊樺木(1x1):147
517. 110033226_ipt_07_磚塊樺木(2x1):148
518. 110033226_ipt_06_磚塊樺木(1x1):148
519. 110033226_ipt_07_磚塊樺木(2x1):149
520. 110033226_ipt_06_磚塊樺木(1x1):149
521. 110033226_ipt_07_磚塊樺木(2x1):150
522. 110033226_ipt_06_磚塊樺木(1x1):150
523. 110033226_ipt_07_磚塊樺木(2x1):151
524. 110033226_ipt_06_磚塊樺木(1x1):151
525. 110033226_ipt_07_磚塊樺木(2x1):152
526. 110033226_ipt_06_磚塊樺木(1x1):152
527. 110033226_ipt_07_磚塊樺木(2x1):153
528. 110033226_ipt_06_磚塊樺木(1x1):153
529. 110033226_ipt_07_磚塊樺木(2x1):154
530. 110033226_ipt_06_磚塊樺木(1x1):154
531. 110033226_ipt_07_磚塊樺木(2x1):155
532. 110033226_ipt_06_磚塊樺木(1x1):155
533. 110033226_ipt_07_磚塊樺木(2x1):156
534. 110033226_ipt_06_磚塊樺木(1x1):160
535. 110033226_ipt_07_磚塊樺木(2x1):161
536. 110033226_ipt_06_磚塊樺木(1x1):161
537. 110033226_ipt_07_磚塊樺木(2x1):162
538. 110033226_ipt_06_磚塊樺木(1x1):162
539. 110033226_ipt_07_磚塊樺木(2x1):163 — 貼合:33
540. 110033226_ipt_06_磚塊樺木(1x1):163
541. 110033226_ipt_07_磚塊樺木(2x1):164
542. 110033226_ipt_06_磚塊樺木(1x1):164
543. 110033226_ipt_07_磚塊樺木(2x1):165 — 貼合:31
544. 110033226_ipt_06_磚塊樺木(1x1):165
545. 110033226_ipt_07_磚塊樺木(2x1):166
546. 110033226_ipt_06_磚塊樺木(1x1):166
547. 110033226_ipt_07_磚塊樺木(2x1):167
548. 110033226_ipt_06_磚塊樺木(1x1):167
549. 110033226_ipt_07_磚塊樺木(2x1):168
550. 110033226_ipt_06_磚塊樺木(1x1):168
551. 110033226_ipt_07_磚塊樺木(2x1):169 — 貼合:35
552. 110033226_ipt_06_磚塊樺木(1x1):169
553. 110033226_ipt_07_磚塊樺木(2x1):170
554. 110033226_ipt_07_磚塊樺木(2x1):3 — 貼合:7, 貼合:8, 貼合:9, 貼合:12
555. 110033226_ipt_06_磚塊樺木(1x1):4 — 貼合:10, 貼合:11, 貼合:12
556. 110033226_ipt_07_磚塊樺木(2x1):6 — 貼合:1, 貼合:2, 貼合:3, 貼合:6, 貼合:7, 貼合:8, 貼合:10, 貼合:11
557. 110033226_ipt_06_磚塊樺木(1x1):5 — 貼合:4, 貼合:5, 貼合:6, 貼合:9
558. 110033226_ipt_07_磚塊樺木(2x1):7
559. 110033226_ipt_06_磚塊樺木(1x1):6
560. 110033226_ipt_07_磚塊樺木(2x1):8
561. 110033226_ipt_06_磚塊樺木(1x1):7
562. 110033226_ipt_07_磚塊樺木(2x1):9
563. 110033226_ipt_06_磚塊樺木(1x1):8
564. 110033226_ipt_07_磚塊樺木(2x1):10
565. 110033226_ipt_06_磚塊樺木(1x1):9
566. 110033226_ipt_07_磚塊樺木(2x1):11
567. 110033226_ipt_06_磚塊樺木(1x1):10
568. 110033226_ipt_07_磚塊樺木(2x1):12
569. 110033226_ipt_06_磚塊樺木(1x1):11
570. 110033226_ipt_07_磚塊樺木(2x1):13
571. 110033226_ipt_06_磚塊樺木(1x1):12
572. 110033226_ipt_07_磚塊樺木(2x1):14
573. 110033226_ipt_06_磚塊樺木(1x1):13
574. 110033226_ipt_07_磚塊樺木(2x1):15
575. 110033226_ipt_06_磚塊樺木(1x1):14
576. 110033226_ipt_07_磚塊樺木(2x1):16
577. 110033226_ipt_06_磚塊樺木(1x1):15
578. 110033226_ipt_07_磚塊樺木(2x1):17
579. 110033226_ipt_06_磚塊樺木(1x1):16
580. 110033226_ipt_07_磚塊樺木(2x1):18
581. 110033226_ipt_06_磚塊樺木(1x1):17
582. 110033226_ipt_07_磚塊樺木(2x1):19
583. 110033226_ipt_06_磚塊樺木(1x1):18
584. 110033226_ipt_07_磚塊樺木(2x1):20
585. 110033226_ipt_06_磚塊樺木(1x1):19
586. 110033226_ipt_07_磚塊樺木(2x1):21 — 貼合:37, 貼合:40
587. 110033226_ipt_06_磚塊樺木(1x1):20
588. 110033226_ipt_07_磚塊樺木(2x1):22
589. 110033226_ipt_06_磚塊樺木(1x1):21
590. 110033226_ipt_07_磚塊樺木(2x1):27
591. 110033226_ipt_06_磚塊樺木(1x1):26
592. 110033226_ipt_07_磚塊樺木(2x1):28
593. 110033226_ipt_06_磚塊樺木(1x1):27
594. 110033226_ipt_07_磚塊樺木(2x1):29
595. 110033226_ipt_06_磚塊樺木(1x1):28
596. 110033226_ipt_07_磚塊樺木(2x1):30
597. 110033226_ipt_06_磚塊樺木(1x1):29
598. 110033226_ipt_07_磚塊樺木(2x1):31
599. 110033226_ipt_06_磚塊樺木(1x1):30
600. 110033226_ipt_07_磚塊樺木(2x1):32
601. 110033226_ipt_06_磚塊樺木(1x1):31
602. 110033226_ipt_07_磚塊樺木(2x1):33
603. 110033226_ipt_06_磚塊樺木(1x1):32
604. 110033226_ipt_07_磚塊樺木(2x1):34
605. 110033226_ipt_06_磚塊樺木(1x1):33
606. 110033226_ipt_07_磚塊樺木(2x1):35
607. 110033226_ipt_06_磚塊樺木(1x1):34
608. 110033226_ipt_07_磚塊樺木(2x1):36
609. 110033226_ipt_06_磚塊樺木(1x1):35
610. 110033226_ipt_07_磚塊樺木(2x1):41
611. 110033226_ipt_06_磚塊樺木(1x1):40
612. 110033226_ipt_07_磚塊樺木(2x1):42
613. 110033226_ipt_06_磚塊樺木(1x1):41
614. 110033226_ipt_07_磚塊樺木(2x1):43
615. 110033226_ipt_06_磚塊樺木(1x1):42
616. 110033226_ipt_07_磚塊樺木(2x1):44
617. 110033226_ipt_06_磚塊樺木(1x1):43
618. 110033226_ipt_07_磚塊樺木(2x1):45
619. 110033226_ipt_06_磚塊樺木(1x1):44
620. 110033226_ipt_07_磚塊樺木(2x1):46
621. 110033226_ipt_06_磚塊樺木(1x1):45
622. 110033226_ipt_07_磚塊樺木(2x1):47
623. 110033226_ipt_06_磚塊樺木(1x1):46
624. 110033226_ipt_07_磚塊樺木(2x1):48
625. 110033226_ipt_06_磚塊樺木(1x1):47
626. 110033226_ipt_07_磚塊樺木(2x1):49
627. 110033226_ipt_06_磚塊樺木(1x1):48
628. 110033226_ipt_07_磚塊樺木(2x1):50
629. 110033226_ipt_06_磚塊樺木(1x1):49
630. 110033226_ipt_07_磚塊樺木(2x1):51
631. 110033226_ipt_06_磚塊樺木(1x1):50 — 貼合:38
632. 110033226_ipt_07_磚塊樺木(2x1):52 — 貼合:39
633. 110033226_ipt_06_磚塊樺木(1x1):51
634. 110033226_ipt_07_磚塊樺木(2x1):53
635. 110033226_ipt_06_磚塊樺木(1x1):52
636. 110033226_ipt_07_磚塊樺木(2x1):54
637. 110033226_ipt_06_磚塊樺木(1x1):53
638. 110033226_ipt_07_磚塊樺木(2x1):55
639. 110033226_ipt_06_磚塊樺木(1x1):54
640. 110033226_ipt_07_磚塊樺木(2x1):56
641. 110033226_ipt_06_磚塊樺木(1x1):55
642. 110033226_ipt_07_磚塊樺木(2x1):57
643. 110033226_ipt_06_磚塊樺木(1x1):56
644. 110033226_ipt_07_磚塊樺木(2x1):58
645. 110033226_ipt_06_磚塊樺木(1x1):57
646. 110033226_ipt_07_磚塊樺木(2x1):59 — 貼合:32
647. 110033226_ipt_06_磚塊樺木(1x1):58
648. 110033226_ipt_07_磚塊樺木(2x1):60
649. 110033226_ipt_06_磚塊樺木(1x1):59
650. 110033226_ipt_07_磚塊樺木(2x1):171
651. 110033226_ipt_06_磚塊樺木(1x1):170
652. 110033226_ipt_07_磚塊樺木(2x1):172 — 貼合:25, 貼合:26, 貼合:27
653. 110033226_ipt_06_磚塊樺木(1x1):171
654. 110033226_ipt_07_磚塊樺木(2x1):173
655. 110033226_ipt_06_磚塊樺木(1x1):172
656. 110033226_ipt_07_磚塊樺木(2x1):174
657. 110033226_ipt_06_磚塊樺木(1x1):173
658. 110033226_ipt_07_磚塊樺木(2x1):175
659. 110033226_ipt_06_磚塊樺木(1x1):174
660. 110033226_ipt_07_磚塊樺木(2x1):176
661. 110033226_ipt_06_磚塊樺木(1x1):175 — 貼合:42
662. 110033226_ipt_07_磚塊樺木(2x1):177
663. 110033226_ipt_06_磚塊樺木(1x1):176
664. 110033226_ipt_07_磚塊樺木(2x1):178
665. 110033226_ipt_06_磚塊樺木(1x1):177
666. 110033226_ipt_07_磚塊樺木(2x1):179
667. 110033226_ipt_06_磚塊樺木(1x1):178
668. 110033226_ipt_07_磚塊樺木(2x1):180
669. 110033226_ipt_06_磚塊樺木(1x1):179
670. 110033226_ipt_07_磚塊樺木(2x1):181
671. 110033226_ipt_06_磚塊樺木(1x1):180
672. 110033226_ipt_07_磚塊樺木(2x1):182
673. 110033226_ipt_06_磚塊樺木(1x1):181
674. 110033226_ipt_07_磚塊樺木(2x1):183
675. 110033226_ipt_06_磚塊樺木(1x1):182
676. 110033226_ipt_07_磚塊樺木(2x1):184
677. 110033226_ipt_06_磚塊樺木(1x1):183
678. 110033226_ipt_07_磚塊樺木(2x1):185
679. 110033226_ipt_06_磚塊樺木(1x1):184
680. 110033226_ipt_07_磚塊樺木(2x1):186
681. 110033226_ipt_06_磚塊樺木(1x1):185
682. 110033226_ipt_07_磚塊樺木(2x1):187
683. 110033226_ipt_06_磚塊樺木(1x1):186
684. 110033226_ipt_07_磚塊樺木(2x1):188
685. 110033226_ipt_06_磚塊樺木(1x1):187
686. 110033226_ipt_07_磚塊樺木(2x1):193
687. 110033226_ipt_06_磚塊樺木(1x1):192
688. 110033226_ipt_07_磚塊樺木(2x1):194
689. 110033226_ipt_06_磚塊樺木(1x1):193
690. 110033226_ipt_07_磚塊樺木(2x1):195
691. 110033226_ipt_06_磚塊樺木(1x1):194
692. 110033226_ipt_07_磚塊樺木(2x1):196
693. 110033226_ipt_06_磚塊樺木(1x1):195
694. 110033226_ipt_07_磚塊樺木(2x1):197
695. 110033226_ipt_06_磚塊樺木(1x1):196
696. 110033226_ipt_07_磚塊樺木(2x1):198
697. 110033226_ipt_06_磚塊樺木(1x1):197
698. 110033226_ipt_07_磚塊樺木(2x1):199
699. 110033226_ipt_06_磚塊樺木(1x1):198
700. 110033226_ipt_07_磚塊樺木(2x1):200
701. 110033226_ipt_06_磚塊樺木(1x1):199
702. 110033226_ipt_07_磚塊樺木(2x1):201 — 貼合:41, 貼合:43
703. 110033226_ipt_06_磚塊樺木(1x1):200
704. 110033226_ipt_07_磚塊樺木(2x1):202
705. 110033226_ipt_06_磚塊樺木(1x1):201
706. 110033226_ipt_07_磚塊樺木(2x1):207
707. 110033226_ipt_06_磚塊樺木(1x1):206
708. 110033226_ipt_07_磚塊樺木(2x1):208
709. 110033226_ipt_06_磚塊樺木(1x1):207
710. 110033226_ipt_07_磚塊樺木(2x1):209
711. 110033226_ipt_06_磚塊樺木(1x1):208
712. 110033226_ipt_07_磚塊樺木(2x1):210
713. 110033226_ipt_06_磚塊樺木(1x1):209
714. 110033226_ipt_07_磚塊樺木(2x1):211
715. 110033226_ipt_06_磚塊樺木(1x1):210
716. 110033226_ipt_07_磚塊樺木(2x1):212
717. 110033226_ipt_06_磚塊樺木(1x1):211
718. 110033226_ipt_07_磚塊樺木(2x1):213
719. 110033226_ipt_06_磚塊樺木(1x1):212
720. 110033226_ipt_07_磚塊樺木(2x1):214 — 貼合:28, 貼合:29
721. 110033226_ipt_06_磚塊樺木(1x1):213 — 貼合:30
722. 110033226_ipt_07_磚塊樺木(2x1):215
723. 110033226_ipt_06_磚塊樺木(1x1):214
724. 110033226_ipt_07_磚塊樺木(2x1):216
725. 110033226_ipt_06_磚塊樺木(1x1):215
726. 110033226_ipt_07_磚塊樺木(2x1):217
727. 110033226_ipt_06_磚塊樺木(1x1):216
728. 110033226_ipt_07_磚塊樺木(2x1):218
729. 110033226_ipt_06_磚塊樺木(1x1):217
730. 110033226_ipt_07_磚塊樺木(2x1):219
731. 110033226_ipt_06_磚塊樺木(1x1):218
732. 110033226_ipt_07_磚塊樺木(2x1):220
733. 110033226_ipt_06_磚塊樺木(1x1):219
734. 110033226_ipt_07_磚塊樺木(2x1):221
735. 110033226_ipt_06_磚塊樺木(1x1):220
736. 110033226_ipt_07_磚塊樺木(2x1):222
737. 110033226_ipt_06_磚塊樺木(1x1):221
738. 110033226_ipt_07_磚塊樺木(2x1):223
739. 110033226_ipt_06_磚塊樺木(1x1):222
740. 110033226_ipt_07_磚塊樺木(2x1):224
741. 110033226_ipt_06_磚塊樺木(1x1):223
742. 110033226_ipt_07_磚塊樺木(2x1):225 — 貼合:34
743. 110033226_ipt_06_磚塊樺木(1x1):224 — 貼合:36
744. 110033226_ipt_07_磚塊樺木(2x1):226
745. 110033226_ipt_06_磚塊樺木(1x1):225
746. 110033226_ipt_08_平滑面(3x1):1 — 貼合:31, 貼合:32, 貼合:33
747. 110033226_ipt_08_平滑面(3x1):4
748. 110033226_ipt_08_平滑面(3x1):5
749. 110033226_ipt_08_平滑面(3x1):6
750. 110033226_ipt_08_平滑面(3x1):7
751. 110033226_ipt_08_平滑面(3x1):8
752. 110033226_ipt_08_平滑面(3x1):9
753. 110033226_ipt_08_平滑面(3x1):10
754. 110033226_ipt_08_平滑面(3x1):18
755. 110033226_ipt_08_平滑面(3x1):19
756. 110033226_ipt_08_平滑面(3x1):20
757. 110033226_ipt_08_平滑面(3x1):21
758. 110033226_ipt_08_平滑面(3x1):22
759. 110033226_ipt_08_平滑面(3x1):23 — 對稱:4, 貼合:168
760. 110033226_ipt_08_平滑面(3x1):24 — 對稱:3
761. 110033226_ipt_08_平滑面(3x1):25
762. 110033226_ipt_08_平滑面(3x1):26
763. 110033226_ipt_08_平滑面(3x1):27
764. 110033226_ipt_08_平滑面(3x1):28
765. 110033226_ipt_08_平滑面(3x1):29
766. 110033226_ipt_08_平滑面(3x1):30
767. 110033226_ipt_08_平滑面(3x1):31
768. 110033226_ipt_08_平滑面(3x1):32
769. 110033226_ipt_08_平滑面(3x1):33
770. 110033226_ipt_08_平滑面(3x1):34
771. 110033226_ipt_08_平滑面(3x1):35 — 貼合:60
772. 110033226_ipt_08_平滑面(3x1):36
773. 110033226_ipt_08_平滑面(3x1):37 — 貼合:63, 貼合:64
774. 110033226_ipt_08_平滑面(3x1):38
775. 110033226_ipt_08_平滑面(3x1):39 — 貼合:59
776. 110033226_ipt_08_平滑面(3x1):40
777. 110033226_ipt_08_平滑面(3x1):41 — 貼合:65
778. 110033226_ipt_08_平滑面(3x1):42
779. 110033226_ipt_08_平滑面(3x1):43 — 貼合:57, 貼合:58
780. 110033226_ipt_08_平滑面(3x1):44
781. 110033226_ipt_08_平滑面(3x1):45
782. 110033226_ipt_08_平滑面(3x1):46
783. 110033226_ipt_08_平滑面(3x1):47
784. 110033226_ipt_08_平滑面(3x1):48 — 貼合:50, 貼合:51, 貼合:53, 貼合:55
785. 110033226_ipt_08_平滑面(3x1):49
786. 110033226_ipt_08_平滑面(3x1):50
787. 110033226_ipt_08_平滑面(3x1):51
788. 110033226_ipt_08_平滑面(3x1):52
789. 110033226_ipt_08_平滑面(3x1):53
790. 110033226_ipt_08_平滑面(3x1):54
791. 110033226_ipt_08_平滑面(3x1):55
792. 110033226_ipt_08_平滑面(3x1):56
793. 110033226_ipt_08_平滑面(3x1):57
794. 110033226_ipt_08_平滑面(3x1):2 — 貼合:34, 貼合:35, 貼合:36
795. 110033226_ipt_08_平滑面(3x1):11
796. 110033226_ipt_08_平滑面(3x1):12 — 貼合:49
797. 110033226_ipt_08_平滑面(3x1):13 — 貼合:44, 貼合:45, 貼合:46, 貼合:47
798. 110033226_ipt_08_平滑面(3x1):14
799. 110033226_ipt_08_平滑面(3x1):15
800. 110033226_ipt_08_平滑面(3x1):16
801. 110033226_ipt_08_平滑面(3x1):17
802. 110033226_ipt_11_樓梯支架:1 — 貼合:63, 貼合:64, 貼合:65, 貼合:66, 貼合:67, 貼合:68
803. 110033226_ipt_11_樓梯支架:2 — 貼合:66, 貼合:67, 貼合:68, 貼合:81
804. 110033226_ipt_11_樓梯支架:6 — 貼合:79
805. 110033226_ipt_11_樓梯支架:7 — 貼合:77
806. 110033226_ipt_11_樓梯支架:8 — 貼合:78
807. 110033226_ipt_11_樓梯支架:9 — 貼合:85
808. 110033226_ipt_11_樓梯支架:10 — 貼合:75, 貼合:82
809. 110033226_ipt_11_樓梯支架:11
810. 110033226_ipt_11_樓梯支架:12 — 貼合:94, 貼合:95
811. 110033226_ipt_11_樓梯支架:13
812. 110033226_ipt_11_樓梯支架:14
813. 110033226_ipt_11_樓梯支架:15
814. 110033226_ipt_11_樓梯支架:16 — 貼合:86, 貼合:87
815. 110033226_ipt_11_樓梯支架:17 — 貼合:84
816. 110033226_ipt_11_樓梯支架:18 — 貼合:83
817. 110033226_ipt_11_樓梯支架:19 — 貼合:70, 貼合:74
818. 110033226_ipt_11_樓梯支架:20 — 貼合:80
819. 110033226_ipt_11_樓梯支架:21 — 貼合:92, 貼合:93
820. 110033226_ipt_11_樓梯支架:22 — 貼合:90, 貼合:91
821. 110033226_ipt_11_樓梯支架:23 — 貼合:88, 貼合:89
822. 110033226_ipt_11_樓梯支架:24
823. 110033226_ipt_11_樓梯支架:25
824. 110033226_ipt_11_樓梯支架:26
825. 110033226_ipt_11_樓梯支架:27 — 貼合:69, 貼合:71, 貼合:73
826. 110033226_ipt_11_樓梯支架:28
827. 110033226_ipt_11_樓梯支架:29
828. 110033226_ipt_11_樓梯支架:30
829. 110033226_ipt_11_樓梯支架:31
830. 110033226_ipt_11_樓梯支架:32
831. 110033226_ipt_11_樓梯支架:33 — 貼合:76
832. 110033226_ipt_11_樓梯支架:34
833. 110033226_ipt_11_樓梯支架:35 — 貼合:72
834. 110033226_ipt_22_塔樓牆壁:1 — 貼合:99, 貼合:100, 貼合:101
835. 110033226_ipt_22_塔樓牆壁:5
836. 110033226_ipt_22_塔樓牆壁:6
837. 110033226_ipt_22_塔樓牆壁:7
838. 110033226_ipt_22_塔樓牆壁:8
839. 110033226_ipt_22_塔樓牆壁:9
840. 110033226_ipt_22_塔樓牆壁:10
841. 110033226_ipt_22_塔樓牆壁:11
842. 110033226_ipt_22_塔樓牆壁:12
843. 110033226_ipt_22_塔樓牆壁:13
844. 110033226_ipt_22_塔樓牆壁:14
845. 110033226_ipt_22_塔樓牆壁:15
846. 110033226_ipt_22_塔樓牆壁:16 — 貼合:105, 貼合:110, 貼合:111, 貼合:112
847. 110033226_ipt_22_塔樓牆壁:17 — 貼合:104
848. 110033226_ipt_22_塔樓牆壁:18
849. 110033226_ipt_22_塔樓牆壁:19 — 貼合:106, 貼合:108
850. 110033226_ipt_22_塔樓牆壁:20 — 貼合:107, 貼合:109
851. 110033226_ipt_22_塔樓牆壁:21 — 貼合:176, 貼合:177
852. 110033226_ipt_22_塔樓牆壁:104 — 貼合:146, 貼合:147, 貼合:148
853. 110033226_ipt_22_塔樓牆壁:105
854. 110033226_ipt_22_塔樓牆壁:106
855. 110033226_ipt_22_塔樓牆壁:107
856. 110033226_ipt_22_塔樓牆壁:108
857. 110033226_ipt_22_塔樓牆壁:109
858. 110033226_ipt_22_塔樓牆壁:110
859. 110033226_ipt_22_塔樓牆壁:111
860. 110033226_ipt_22_塔樓牆壁:112
861. 110033226_ipt_22_塔樓牆壁:113
862. 110033226_ipt_22_塔樓牆壁:114
863. 110033226_ipt_22_塔樓牆壁:115
864. 110033226_ipt_22_塔樓牆壁:116
865. 110033226_ipt_22_塔樓牆壁:117
866. 110033226_ipt_22_塔樓牆壁:118
867. 110033226_ipt_22_塔樓牆壁:119
868. 110033226_ipt_22_塔樓牆壁:120
869. 110033226_ipt_22_塔樓牆壁:121
870. 110033226_ipt_22_塔樓牆壁:122
871. 110033226_ipt_22_塔樓牆壁:123
872. 110033226_ipt_22_塔樓牆壁:124
873. 110033226_ipt_22_塔樓牆壁:125
874. 110033226_ipt_22_塔樓牆壁:126
875. 110033226_ipt_22_塔樓牆壁:127
876. 110033226_ipt_22_塔樓牆壁:128
877. 110033226_ipt_22_塔樓牆壁:129 — 貼合:154, 貼合:155
878. 110033226_ipt_22_塔樓牆壁:130
879. 110033226_ipt_22_塔樓牆壁:131
880. 110033226_ipt_22_塔樓牆壁:132
881. 110033226_ipt_22_塔樓牆壁:133
882. 110033226_ipt_22_塔樓牆壁:134
883. 110033226_ipt_22_塔樓牆壁:135 — 貼合:156, 貼合:157, 貼合:158
884. 110033226_ipt_22_塔樓牆壁:136
885. 110033226_ipt_22_塔樓牆壁:137 — 貼合:159
886. 110033226_ipt_22_塔樓牆壁:138
887. 110033226_ipt_22_塔樓牆壁:139
888. 110033226_ipt_22_塔樓牆壁:146 — 貼合:157, 貼合:158, 貼合:159
889. 110033226_ipt_22_塔樓牆壁:163
890. 110033226_ipt_22_塔樓牆壁:164
891. 110033226_ipt_22_塔樓牆壁:165
892. 110033226_ipt_22_塔樓牆壁:166
893. 110033226_ipt_22_塔樓牆壁:167
894. 110033226_ipt_22_塔樓牆壁:168
895. 110033226_ipt_22_塔樓牆壁:169
896. 110033226_ipt_22_塔樓牆壁:170
897. 110033226_ipt_22_塔樓牆壁:171
898. 110033226_ipt_22_塔樓牆壁:172
899. 110033226_ipt_22_塔樓牆壁:173
900. 110033226_ipt_22_塔樓牆壁:174
901. 110033226_ipt_22_塔樓牆壁:175
902. 110033226_ipt_22_塔樓牆壁:176
903. 110033226_ipt_22_塔樓牆壁:177
904. 110033226_ipt_22_塔樓牆壁:178
905. 110033226_ipt_22_塔樓牆壁:179
906. 110033226_ipt_22_塔樓牆壁:180
907. 110033226_ipt_22_塔樓牆壁:181
908. 110033226_ipt_22_塔樓牆壁:182
909. 110033226_ipt_22_塔樓牆壁:183
910. 110033226_ipt_22_塔樓牆壁:184
911. 110033226_ipt_22_塔樓牆壁:185
912. 110033226_ipt_22_塔樓牆壁:186
913. 110033226_ipt_22_塔樓牆壁:187
914. 110033226_ipt_22_塔樓牆壁:188
915. 110033226_ipt_22_塔樓牆壁:189
916. 110033226_ipt_22_塔樓牆壁:190
917. 110033226_ipt_22_塔樓牆壁:191
918. 110033226_ipt_22_塔樓牆壁:192 — 貼合:160, 貼合:161, 貼合:162
919. 110033226_ipt_22_塔樓牆壁:195
920. 110033226_ipt_22_塔樓牆壁:196
921. 110033226_ipt_22_塔樓牆壁:197
922. 110033226_ipt_22_塔樓牆壁:198
923. 110033226_ipt_22_塔樓牆壁:199
924. 110033226_ipt_22_塔樓牆壁:200
925. 110033226_ipt_22_塔樓牆壁:201
926. 110033226_ipt_22_塔樓牆壁:202
927. 110033226_ipt_22_塔樓牆壁:203
928. 110033226_ipt_22_塔樓牆壁:204
929. 110033226_ipt_22_塔樓牆壁:205
930. 110033226_ipt_10_木板條:2 — 貼合:110, 貼合:111, 貼合:112
931. 110033226_ipt_10_木板條:4
932. 110033226_ipt_10_木板條:5
933. 110033226_ipt_10_木板條:6
934. 110033226_ipt_10_木板條:7
935. 110033226_ipt_10_木板條:8
936. 110033226_ipt_10_木板條:9
937. 110033226_ipt_10_木板條:10
938. 110033226_ipt_10_木板條:11
939. 110033226_ipt_10_木板條:12
940. 110033226_ipt_10_木板條:13
941. 110033226_ipt_10_木板條:14
942. 110033226_ipt_10_木板條:15
943. 110033226_ipt_10_木板條:16
944. 110033226_ipt_10_木板條:17
945. 110033226_ipt_10_木板條:18
946. 110033226_ipt_10_木板條:19
947. 110033226_ipt_10_木板條:20
948. 110033226_ipt_10_木板條:21
949. 110033226_ipt_10_木板條:22
950. 110033226_ipt_10_木板條:23
951. 110033226_ipt_10_木板條:24
952. 110033226_ipt_10_木板條:25
953. 110033226_ipt_10_木板條:26
954. 110033226_ipt_10_木板條:27
955. 110033226_ipt_10_木板條:28
956. 110033226_ipt_10_木板條:29 — 貼合:117
957. 110033226_ipt_10_木板條:30 — 貼合:115
958. 110033226_ipt_10_木板條:31 — 貼合:116
959. 110033226_ipt_10_木板條:32
960. 110033226_ipt_10_木板條:46
961. 110033226_ipt_10_木板條:47
962. 110033226_ipt_10_木板條:48
963. 110033226_ipt_10_木板條:49
964. 110033226_ipt_10_木板條:50
965. 110033226_ipt_10_木板條:51
966. 110033226_ipt_10_木板條:52
967. 110033226_ipt_10_木板條:53
968. 110033226_ipt_10_木板條:54
969. 110033226_ipt_10_木板條:55
970. 110033226_ipt_10_木板條:56
971. 110033226_ipt_10_木板條:57
972. 110033226_ipt_10_木板條:58
973. 110033226_ipt_10_木板條:59
974. 110033226_ipt_10_木板條:60
975. 110033226_ipt_10_木板條:61
976. 110033226_ipt_10_木板條:62
977. 110033226_ipt_10_木板條:63
978. 110033226_ipt_10_木板條:64
979. 110033226_ipt_10_木板條:65
980. 110033226_ipt_10_木板條:66
981. 110033226_ipt_10_木板條:67
982. 110033226_ipt_10_木板條:68
983. 110033226_ipt_10_木板條:69
984. 110033226_ipt_10_木板條:70
985. 110033226_ipt_10_木板條:71
986. 110033226_ipt_10_木板條:72